# Autodesk Inventor assembly: Assembly1
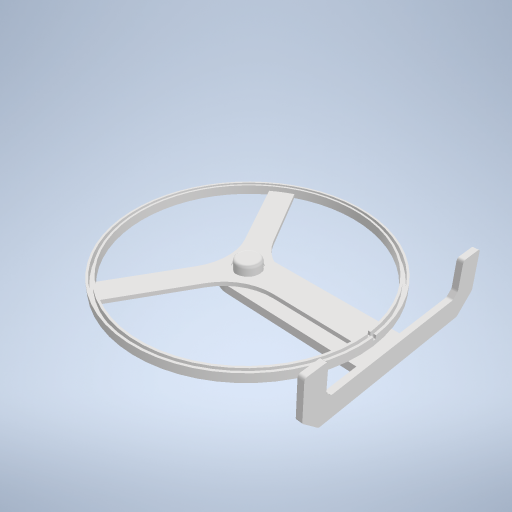
[picture p0: Inventor's stored thumbnail of the model, 512x512]
Saved by Autodesk Inventor 2023 (Build 270158000, 158)
## iProperties
Created: 2023-09-22
Part Number: Assembly1
Document SubType Name: Assembly
Designer: vlada
Author: vlada
## Documents named in this file (3)
- C:\Users\vlada\OneDrive\Plocha\leuze\3D\Assembly1.iam
- C:\Users\vlada\OneDrive\Plocha\projekty\Inventor\vt2020\PaperHolder.ipt
- C:\Users\vlada\OneDrive\Plocha\leuze\3D\Holder.ipt
## Components (2 placed, 2 different names)
1. PaperHolder:1 — Flush:1
2. Holder:1 — Flush:1
## Relationships (1: Flush 1)
- Flush:1: PaperHolder:1 ↔ Holder:1
